# Autodesk Inventor assembly: ASY MSC 010 cone
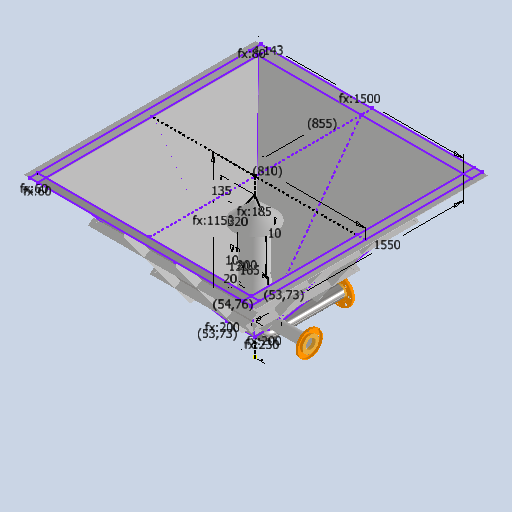
[picture p0: Inventor's stored thumbnail of the model, 512x512]
Saved by Autodesk Inventor 2025 (Build 290162010, 162A)
## iProperties
Created: 2024-05-19
Part Number: ASY MSC 010 cone
Document SubType Name: Assembly
Designer: admin
Mass: 216247 g
Surface Area: 140674 cm^2
Volume: 27030.8 cm^3
Density: 8 g/cm^3
Stock Number: ASY МОО 010 конус
Author: admin
## Documents named in this file (17)
- C:\Users\DELL\YandexDisk-badmisterfox\домашниий пк\Inventor\Manturovo\Manturovo_Se-clar\ASY MSC 010 cone.iam
- C:\Users\DELL\YandexDisk-badmisterfox\домашниий пк\Inventor\Manturovo\Manturovo_Se-clar\конус\MSC 014 cone IN right board.ipt
- C:\Users\DELL\YandexDisk-badmisterfox\домашниий пк\Inventor\Manturovo\Manturovo_Se-clar\конус\MSC 011 cone IN bottom.ipt
- C:\Users\DELL\YandexDisk-badmisterfox\домашниий пк\Inventor\Manturovo\Manturovo_Se-clar\конус\MSC 013 cone IN left board.ipt
- C:\Users\DELL\YandexDisk-badmisterfox\домашниий пк\Inventor\Manturovo\Manturovo_Se-clar\конус\MSC 012 cone IN back.ipt
- C:\Users\DELL\YandexDisk-badmisterfox\домашниий пк\Inventor\Manturovo\Manturovo_Se-clar\конус\MSC 019 cone sketch.ipt
- C:\Users\DELL\YandexDisk-badmisterfox\домашниий пк\Inventor\Manturovo\Manturovo_Se-clar\конус\MSC 015 cone IN bow.ipt
- C:\Users\DELL\YandexDisk-badmisterfox\домашниий пк\Inventor\Manturovo\Manturovo_Se-clar\MSC 0691 stringer cone.ipt
- C:\Users\DELL\YandexDisk-badmisterfox\домашниий пк\Inventor\Manturovo\Manturovo_Se-clar\MSC 0561 rib cone.ipt
- C:\Users\DELL\YandexDisk-badmisterfox\домашниий пк\Inventor\Manturovo\Manturovo_Se-clar\MSC 0562 rib cone.ipt
- C:\Users\DELL\YandexDisk-badmisterfox\домашниий пк\Inventor\Manturovo\Manturovo_Se-clar\MSC 0563 rib cone.ipt
- C:\Users\DELL\YandexDisk-badmisterfox\домашниий пк\Inventor\Manturovo\Manturovo_Se-clar\MSC 0564 rib cone.ipt
- C:\Users\DELL\YandexDisk-badmisterfox\домашниий пк\Inventor\Manturovo\Manturovo_Se-clar\ASY MSC 300 Cone tube.iam
- C:\Users\DELL\YandexDisk-badmisterfox\домашниий пк\Inventor\Manturovo\Manturovo_Se-clar\ASY MSC 080 roсket.iam
- C:\Users\DELL\YandexDisk-badmisterfox\домашниий пк\Inventor\Manturovo\Manturovo_Se-clar\ракета\МОО 068 ракета труба 8.ipt
- C:\Users\admin\YandexDisk-badmisterfox\домашниий пк\Inventor\Manturovo\Manturovo_Se-clar\3d party\Stamp flange DIN2642\Stamd flange lapped collar DIN2642.ipt
- C:\Users\DELL\YandexDisk-badmisterfox\домашниий пк\Inventor\Manturovo\Manturovo_Se-clar\3d party\Stamp flange DIN2642\Stamd flange lapped collar DIN2642\Stamp flange DIN2642-065.ipt
## Components (26 placed, 15 different names)
1. MSC 019 cone sketch.ipt:1 — Flush:8, Flush:9, Mate:1
2. MSC 012 cone IN back.ipt:1 — Flush:6, Flush:10, Mate:2, Flush:12, Mate:38, Mate:49, Mate:51, Mate:52, Mate:55, Mate:58
3. MSC 011 cone IN bottom.ipt:1 — Flush:4, Flush:5, Flush:11, Rigid:1
4. MSC 014 cone IN right board.ipt:1 — Flush:12, Flush:13, Flush:15, Mate:28, Mate:39, Mate:63, Mate:66
5. MSC 013 cone IN left board.ipt:1 — Mate:4, Flush:14, Mate:5
6. MSC 015 cone IN bow.ipt:1 — Mate:3, Mate:6, Flush:16, Flush:17
7. ASY MSC 300 Cone tube:1 [sub-assembly] — Rigid:1, Rigid:2
8. ASY MSC 080 roсket.iam:1 [sub-assembly] — Rigid:2
9. МОО 068 ракета труба 8:1 — Rigid:3
10. Stamp flange DIN2642-065:1 — Rigid:3
11. MSC 0691 stringer cone:3 — Mate:49, Mate:50, Mate:51, Mate:54, Mate:56, Mate:57, Mate:59, Mate:60
12. MSC 0691 stringer cone:5 — Mate:52, Mate:53, Mate:54
13. MSC 0561 rib cone:1 — Mate:55, Mate:56, Mate:57
14. MSC 0562 rib cone:1 — Mate:58, Mate:59, Mate:60
15. MSC 0691 stringer cone:4 — Mate:28, Mate:43, Mate:62, Mate:64, Mate:65, Mate:67, Mate:68
16. MSC 0563 rib cone:1 — Mate:66, Mate:67, Mate:68
17. MSC 0564 rib cone:1 — Mate:63, Mate:64, Mate:65
18. MSC 0691 stringer cone:2 — Mate:38, Mate:39, Mate:43, Mate:61
19. MSC 0691 stringer cone:6
20. MSC 0691 stringer cone:7
21. MSC 0561 rib cone:2
22. MSC 0562 rib cone:2
23. MSC 0691 stringer cone:8
24. MSC 0563 rib cone:2
25. MSC 0564 rib cone:2
26. MSC 0691 stringer cone:9
## Component patterns: (2 elements, first: MSC 0691 stringer cone:3 + MSC 0691 stringer cone:5 + MSC 0561 rib cone:1 + MSC 0562 rib cone:1 + MSC 0691 stringer cone:4 + MSC 0563 rib cone:1 + MSC 0564 rib cone:1 + MSC 0691 stringer cone:2)
## Relationships (47: Mate 30, Flush 13, WeldJoint 3, CylindricalJoint 1)
- Flush:4: MSC 011 cone IN bottom.ipt:1
- Flush:5: MSC 011 cone IN bottom.ipt:1
- Flush:6: MSC 012 cone IN back.ipt:1
- Flush:8: MSC 019 cone sketch.ipt:1
- Flush:9: MSC 019 cone sketch.ipt:1
- Mate:1: MSC 019 cone sketch.ipt:1
- Flush:10: MSC 012 cone IN back.ipt:1
- Mate:2: MSC 012 cone IN back.ipt:1
- Flush:11 (-230 mm): MSC 011 cone IN bottom.ipt:1
- Mate:3: MSC 015 cone IN bow.ipt:1
- Flush:12: MSC 012 cone IN back.ipt:1 ↔ MSC 014 cone IN right board.ipt:1
- Flush:13: MSC 014 cone IN right board.ipt:1
- Mate:4: MSC 013 cone IN left board.ipt:1
- Flush:14: MSC 013 cone IN left board.ipt:1
- Mate:5: MSC 013 cone IN left board.ipt:1
- Flush:15: MSC 014 cone IN right board.ipt:1
- Mate:6: MSC 015 cone IN bow.ipt:1
- Flush:16: MSC 015 cone IN bow.ipt:1
- Flush:17: MSC 015 cone IN bow.ipt:1
- Mate:28: MSC 014 cone IN right board.ipt:1 ↔ MSC 0691 stringer cone:4
- Mate:38 (188.5 mm): MSC 012 cone IN back.ipt:1 ↔ MSC 0691 stringer cone:2
- Mate:39: MSC 014 cone IN right board.ipt:1 ↔ MSC 0691 stringer cone:2
- Mate:43 (377 mm): MSC 0691 stringer cone:4 ↔ MSC 0691 stringer cone:2
- Mate:49: MSC 012 cone IN back.ipt:1 ↔ MSC 0691 stringer cone:3
- Mate:50 (390 mm): MSC 0691 stringer cone:3
- Mate:51 (188.5 mm): MSC 012 cone IN back.ipt:1 ↔ MSC 0691 stringer cone:3
- Mate:52: MSC 012 cone IN back.ipt:1 ↔ MSC 0691 stringer cone:5
- Mate:53 (390 mm): MSC 0691 stringer cone:5
- Mate:54 (377 mm): MSC 0691 stringer cone:3 ↔ MSC 0691 stringer cone:5
- Mate:55: MSC 012 cone IN back.ipt:1 ↔ MSC 0561 rib cone:1
- Mate:56: MSC 0691 stringer cone:3 ↔ MSC 0561 rib cone:1
- Mate:57: MSC 0691 stringer cone:3 ↔ MSC 0561 rib cone:1
- Mate:58: MSC 012 cone IN back.ipt:1 ↔ MSC 0562 rib cone:1
- Mate:59: MSC 0691 stringer cone:3 ↔ MSC 0562 rib cone:1
- Mate:60: MSC 0691 stringer cone:3 ↔ MSC 0562 rib cone:1
- Mate:61 (390 mm): MSC 0691 stringer cone:2
- Mate:62 (390 mm): MSC 0691 stringer cone:4
- Mate:63: MSC 014 cone IN right board.ipt:1 ↔ MSC 0564 rib cone:1
- Mate:64: MSC 0691 stringer cone:4 ↔ MSC 0564 rib cone:1
- Mate:65: MSC 0691 stringer cone:4 ↔ MSC 0564 rib cone:1
- Mate:66: MSC 014 cone IN right board.ipt:1 ↔ MSC 0563 rib cone:1
- Mate:67: MSC 0691 stringer cone:4 ↔ MSC 0563 rib cone:1
- Mate:68: MSC 0691 stringer cone:4 ↔ MSC 0563 rib cone:1
- Rigid:1 [WeldJoint]: MSC 011 cone IN bottom.ipt:1 ↔ ASY MSC 300 Cone tube:1
- Rigid:2 [WeldJoint] (50 mm): ASY MSC 300 Cone tube:1 ↔ ASY MSC 080 roсket.iam:1
- [CylindricalJoint]: MSC 013 cone IN left board.ipt:1 ↔ МОО 068 ракета труба 8:1
- Rigid:3 [WeldJoint]: МОО 068 ракета труба 8:1 ↔ Stamp flange DIN2642-065:1
